# Autodesk Inventor assembly: Förderband
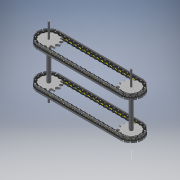
[picture p0: Inventor's stored thumbnail of the model, 180x180]
Saved by Autodesk Inventor 2018 (Build 220112000, 112)
## iProperties
Created: 2018-01-11
Part Number: Förderband
Material: Generisch
Document SubType Name: Assembly
Designer: Dominik
Author: Dominik
## Documents named in this file (5)
- C:\Users\Dominik\Desktop\Diplomarbeit\fuettr_prototype\Mechanical\Inventorskizzen\Förderband.iam
- C:\Users\Dominik\Desktop\Diplomarbeit\fuettr_prototype\Mechanical\Inventorskizzen\Kettenradzusammensetzung_fertig.iam
- C:\Users\Dominik\Desktop\Diplomarbeit\fuettr_prototype\Mechanical\Inventorskizzen\Kettenradzusammensetzung_links.iam
- C:\Users\Dominik\Desktop\Diplomarbeit\fuettr_prototype\Mechanical\Inventorskizzen\Förderbandwelle_vorne.ipt
- C:\Users\Dominik\Desktop\Diplomarbeit\fuettr_prototype\Mechanical\Inventorskizzen\Förderbandwelle_hinten.ipt
## Components (4 placed, 4 different names)
1. Kettenradzusammensetzung_fertig:1 [sub-assembly] — Passend:3, Passend:4, Passend:6
2. Kettenradzusammensetzung_links:1 [sub-assembly] — Passend:1, Passend:2, Passend:5
3. Förderbandwelle_vorne:1 — Passend:5, Passend:6
4. Förderbandwelle_hinten:1 — Passend:1, Passend:2, Passend:3, Passend:4
## Relationships (6: Mate 6)
- Passend:1 [Mate]: Kettenradzusammensetzung_links:1 ↔ Förderbandwelle_hinten:1
- Passend:2 [Mate]: Kettenradzusammensetzung_links:1 ↔ Förderbandwelle_hinten:1
- Passend:3 [Mate]: Kettenradzusammensetzung_fertig:1 ↔ Förderbandwelle_hinten:1
- Passend:4 [Mate]: Kettenradzusammensetzung_fertig:1 ↔ Förderbandwelle_hinten:1
- Passend:5 [Mate]: Kettenradzusammensetzung_links:1 ↔ Förderbandwelle_vorne:1
- Passend:6 [Mate]: Kettenradzusammensetzung_fertig:1 ↔ Förderbandwelle_vorne:1
